# Autodesk Inventor assembly: Сборка1
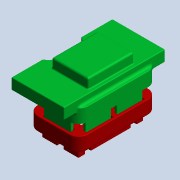
[picture p0: Inventor's stored thumbnail of the model, 180x180]
Saved by Autodesk Inventor 2020 (Build 240168000, 168)
## iProperties
Part Number: Сборка1
Document SubType Name: Сборка
Designer: User
Author: User
## Documents named in this file (3)
- C:\Users\User\Desktop\Project\Test Motion 2\Сборка1.iam
- C:\Users\User\Desktop\Project\Test Motion 2\Main_v2.ipt
- C:\Users\User\Desktop\Project\Test Motion 2\Motion_v2.ipt
## Components (2 placed, 2 different names)
1. Main_v2:1 — Совмещение:1, Совмещение:2, Совмещение:3, Совмещение:4, Совмещение:5
2. Motion_v2:1 — Совмещение:6, Совмещение:7, Совмещение:8
## Relationships (8: Mate 8)
- Совмещение:1 [Mate]: Main_v2:1
- Совмещение:2 [Mate]: Main_v2:1
- Совмещение:3 [Mate]: Main_v2:1
- Совмещение:4 [Mate]: Main_v2:1
- Совмещение:5 [Mate]: Main_v2:1
- Совмещение:6 [Mate]: Motion_v2:1
- Совмещение:7 [Mate]: Motion_v2:1
- Совмещение:8 [Mate]: Motion_v2:1
